# Autodesk Inventor assembly: Trunk
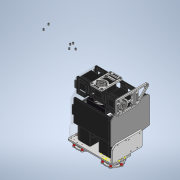
[picture p0: Inventor's stored thumbnail of the model, 180x180]
Saved by Autodesk Inventor 2020.4 (Build 244396000, 396)
## iProperties
Created: 2021-09-10
Part Number: Trunk
Document SubType Name: Assembly
Designer: Masato
Mass: 1170.41 g
Surface Area: 3693.43 cm^2
Volume: 659.985 cm^3
Density: 1.77338 g/cm^3
Author: Masato
## Documents named in this file (20)
- C:\Users\Masato\Documents\Inventor\CIT Brains_Inventor\OpenPlatform_ver3_0 - ve4_1 branch\UpperBody\Trunk\Trunk.iam
- C:\Users\Masato\Documents\Inventor\CIT Brains_Inventor\OpenPlatform_ver3_0 - ve4_1 branch\Ready_Made\KONDO\B3M-SC-1170-A.ipt
- C:\Users\Masato\Documents\Inventor\CIT Brains_Inventor\OpenPlatform_ver3_0 - ve4_1 branch\Ready_Made\KONDO\B3M-SC-1040-A.ipt
- C:\Users\Masato\Documents\Inventor\CIT Brains_Inventor\OpenPlatform_ver3_0 - ve4_1 branch\Ready_Made\Screw\M2_6-15.ipt
- C:\Users\Masato\Documents\Inventor\CIT Brains_Inventor\OpenPlatform_ver3_0 - ve4_1 branch\Ready_Made\KONDO\ClampHorn_Screw.ipt
- C:\Users\Masato\Documents\Inventor\CIT Brains_Inventor\OpenPlatform_ver3_0 - ve4_1 branch\Ready_Made\KONDO\ClampHorn.ipt
- C:\Users\Masato\Documents\Inventor\CIT Brains_Inventor\OpenPlatform_ver3_0 - ve4_1 branch\Ready_Made\Jetson_Xavier_NX_DevKit_without_Wi-FiAntennas\Jetson_Xavier_NX_DevKit.ipt
- C:\Users\Masato\Documents\Inventor\CIT Brains_Inventor\OpenPlatform_ver3_0 - ve4_1 branch\UpperBody\Trunk\Trunk_waisit_frame_.ipt
- C:\Users\Masato\Documents\Inventor\CIT Brains_Inventor\OpenPlatform_ver3_0 - ve4_1 branch\UpperBody\Trunk\CrossRollerBearing\BearingUnit.iam
- C:\Users\Masato\Documents\Inventor\CIT Brains_Inventor\OpenPlatform_ver3_0 - ve4_1 branch\Ready_Made\HP-G830C2800S3.ipt
- C:\Users\Masato\Documents\Inventor\CIT Brains_Inventor\OpenPlatform_ver3_0 - ve4_1 branch\UpperBody\Trunk\Trunk_upper_side_frame.ipt
- C:\Users\Masato\Documents\Inventor\CIT Brains_Inventor\OpenPlatform_ver3_0 - ve4_1 branch\UpperBody\Trunk\Trunk_chest_frame.ipt
- C:\Users\Masato\Documents\Inventor\CIT Brains_Inventor\OpenPlatform_ver3_0 - ve4_1 branch\UpperBody\Trunk\Trunk_lower_side_frame.ipt
- C:\Users\Masato\Documents\Inventor\CIT Brains_Inventor\OpenPlatform_ver3_0 - ve4_1 branch\UpperBody\Trunk\Trunk_shoulder_frame_.ipt
- C:\Users\Masato\Documents\Inventor\CIT Brains_Inventor\OpenPlatform_ver3_0 - ve4_1 branch\UpperBody\Trunk\Trunk_neck_Upper_frame.ipt
- C:\Users\Masato\Documents\Inventor\CIT Brains_Inventor\OpenPlatform_ver3_0 - ve4_1 branch\Ready_Made\InsertNut\IRU-304SW.ipt
- C:\Users\Masato\Documents\Inventor\CIT Brains_Inventor\OpenPlatform_ver3_0 - ve4_1 branch\Ready_Made\Screw\M3-8.ipt
- C:\Users\Masato\Documents\Inventor\CIT Brains_Inventor\OpenPlatform_ver3_0 - ve4_1 branch\UpperBody\Cockpit\Cockpit_side_frame.ipt
- C:\Users\Masato\Documents\Inventor\CIT Brains_Inventor\OpenPlatform_ver3_0 - ve4_1 branch\UpperBody\Cockpit\Cockpit_front_frame.ipt
- ClampHorn.ipt
## Components (48 placed, 19 different names)
1. B3M11xx:3 — 挿入:681, 挿入:686, 挿入:721, 挿入:722
2. B3M-SC-1040-A:4 — 挿入:679, 挿入:684, 挿入:717, 挿入:718, フラッシュ:2, フラッシュ:3
3. B3M-SC-1040-A:5 — 挿入:680, 挿入:685, フラッシュ:2, フラッシュ:3
4. ClampHorn_Screw:3 — 挿入:684
5. ClampHorn_Screw:4 — 挿入:685
6. ClampHorn_Screw:5 — 挿入:686
7. ClampHorn:3 — 挿入:679
8. ClampHorn:4 — 挿入:680
9. ClampHorn:5 — 挿入:681
10. B3M-SC-1170-A:1 — 挿入:689, 挿入:690
11. B3M-SC-1170-A:2 — 挿入:687, 挿入:688
12. Jetson_Xavier_NX_DevKit:1 — フラッシュ:5, フラッシュ:6, メイト:8
13. Trunk_waisit_frame_:1 — フラッシュ:1, 挿入:687, 挿入:688, 挿入:689, 挿入:690, 挿入:693, 挿入:694, 挿入:695, 挿入:696, メイト:5, 挿入:709, 挿入:710, 挿入:711, 挿入:712
14. BearingUnit:1 [sub-assembly] — 挿入:694, 挿入:695
15. BearingUnit:2 [sub-assembly] — 挿入:693, 挿入:696
16. HP-G830C2800S3:1
17. Trunk_upper_side_frame:1 — 挿入:699, 挿入:700, 挿入:713, 挿入:714, 挿入:715, 挿入:716, 挿入:741, 挿入:742, フラッシュ:4, メイト:6
18. Trunk_upper_side_frame:2 — 挿入:701, 挿入:702
19. Trunk_chest_frame:1 — 挿入:699, 挿入:700, 挿入:701, 挿入:702, 挿入:719, 挿入:733, 挿入:734, 挿入:735, 挿入:736, 挿入:737, 挿入:738, 挿入:739, 挿入:740, メイト:7
20. Trunk_lower_side_frame:1 — 挿入:709, 挿入:710, 挿入:713, 挿入:714
21. Trunk_lower_side_frame:2 — 挿入:711, 挿入:712
22. Trunk_shoulder_frame_:1 — 挿入:715, 挿入:716, 挿入:717, 挿入:718
23. Trunk_neck_Upper_frame:1 — 挿入:719, 挿入:721, 挿入:722, 挿入:727, 挿入:728, 挿入:729, 挿入:730, 挿入:731, 挿入:732, 挿入:743, 挿入:744
24. IRU-304SW:1 — 挿入:733
25. IRU-304SW:2 — 挿入:734
26. IRU-304SW:3 — 挿入:735
27. IRU-304SW:4 — 挿入:736
28. IRU-304SW:5 — 挿入:737
29. IRU-304SW:6 — 挿入:738
30. IRU-304SW:7 — 挿入:739
31. IRU-304SW:8 — 挿入:740
32. IRU-304SW:10
33. IRU-304SW:11
34. M3-8:1 — 挿入:728
35. M3-8:2 — 挿入:743
36. M3-8:3 — 挿入:744
37. M3-8:4 — 挿入:727
38. M2_6-15:13 — 挿入:729
39. M2_6-15:14 — 挿入:730
40. M2_6-15:15 — 挿入:731
41. M2_6-15:16 — 挿入:732
42. IRU-304SW:13
43. IRU-304SW:14
44. IRU-304SW:15
45. IRU-304SW:16
46. Trunk_chest_frame:2 — 挿入:741, 挿入:742
47. Cockpit_side_frame:1 — フラッシュ:4, メイト:6, メイト:7, フラッシュ:5, フラッシュ:6, メイト:8, 挿入:745
48. Cockpit_front_frame:1 — 挿入:745
## Relationships (60: Insert 50, Flush 6, Mate 4)
- 挿入:679 [Insert]: B3M-SC-1040-A:4 ↔ ClampHorn:3
- 挿入:680 [Insert]: B3M-SC-1040-A:5 ↔ ClampHorn:4
- 挿入:681 [Insert]: B3M11xx:3 ↔ ClampHorn:5
- 挿入:684 [Insert]: B3M-SC-1040-A:4 ↔ ClampHorn_Screw:3
- 挿入:685 [Insert]: B3M-SC-1040-A:5 ↔ ClampHorn_Screw:4
- 挿入:686 [Insert]: B3M11xx:3 ↔ ClampHorn_Screw:5
- フラッシュ:1 [Flush]: Trunk_waisit_frame_:1
- 挿入:687 [Insert]: B3M-SC-1170-A:2 ↔ Trunk_waisit_frame_:1
- 挿入:688 [Insert]: B3M-SC-1170-A:2 ↔ Trunk_waisit_frame_:1
- 挿入:689 [Insert]: B3M-SC-1170-A:1 ↔ Trunk_waisit_frame_:1
- 挿入:690 [Insert]: B3M-SC-1170-A:1 ↔ Trunk_waisit_frame_:1
- 挿入:693 [Insert]: Trunk_waisit_frame_:1 ↔ BearingUnit:2
- 挿入:694 [Insert]: Trunk_waisit_frame_:1 ↔ BearingUnit:1
- 挿入:695 [Insert]: Trunk_waisit_frame_:1 ↔ BearingUnit:1
- 挿入:696 [Insert]: Trunk_waisit_frame_:1 ↔ BearingUnit:2
- メイト:5 [Mate]: Trunk_waisit_frame_:1
- 挿入:699 [Insert]: Trunk_upper_side_frame:1 ↔ Trunk_chest_frame:1
- 挿入:700 [Insert]: Trunk_upper_side_frame:1 ↔ Trunk_chest_frame:1
- 挿入:701 [Insert]: Trunk_upper_side_frame:2 ↔ Trunk_chest_frame:1
- 挿入:702 [Insert]: Trunk_upper_side_frame:2 ↔ Trunk_chest_frame:1
- 挿入:709 [Insert]: Trunk_waisit_frame_:1 ↔ Trunk_lower_side_frame:1
- 挿入:710 [Insert]: Trunk_waisit_frame_:1 ↔ Trunk_lower_side_frame:1
- 挿入:711 [Insert]: Trunk_waisit_frame_:1 ↔ Trunk_lower_side_frame:2
- 挿入:712 [Insert]: Trunk_waisit_frame_:1 ↔ Trunk_lower_side_frame:2
- 挿入:713 [Insert]: Trunk_upper_side_frame:1 ↔ Trunk_lower_side_frame:1
- 挿入:714 [Insert]: Trunk_upper_side_frame:1 ↔ Trunk_lower_side_frame:1
- 挿入:715 [Insert]: Trunk_upper_side_frame:1 ↔ Trunk_shoulder_frame_:1
- 挿入:716 [Insert]: Trunk_upper_side_frame:1 ↔ Trunk_shoulder_frame_:1
- 挿入:717 [Insert]: B3M-SC-1040-A:4 ↔ Trunk_shoulder_frame_:1
- 挿入:718 [Insert]: B3M-SC-1040-A:4 ↔ Trunk_shoulder_frame_:1
- 挿入:719 [Insert]: Trunk_chest_frame:1 ↔ Trunk_neck_Upper_frame:1
- 挿入:721 [Insert]: B3M11xx:3 ↔ Trunk_neck_Upper_frame:1
- 挿入:722 [Insert]: B3M11xx:3 ↔ Trunk_neck_Upper_frame:1
- 挿入:727 [Insert]: Trunk_neck_Upper_frame:1 ↔ M3-8:4
- 挿入:728 [Insert]: Trunk_neck_Upper_frame:1 ↔ M3-8:1
- 挿入:729 [Insert]: Trunk_neck_Upper_frame:1 ↔ M2_6-15:13
- 挿入:730 [Insert]: Trunk_neck_Upper_frame:1 ↔ M2_6-15:14
- 挿入:731 [Insert]: Trunk_neck_Upper_frame:1 ↔ M2_6-15:15
- 挿入:732 [Insert]: Trunk_neck_Upper_frame:1 ↔ M2_6-15:16
- 挿入:733 [Insert]: Trunk_chest_frame:1 ↔ IRU-304SW:1
- 挿入:734 [Insert]: Trunk_chest_frame:1 ↔ IRU-304SW:2
- 挿入:735 [Insert]: Trunk_chest_frame:1 ↔ IRU-304SW:3
- 挿入:736 [Insert]: Trunk_chest_frame:1 ↔ IRU-304SW:4
- 挿入:737 [Insert]: Trunk_chest_frame:1 ↔ IRU-304SW:5
- 挿入:738 [Insert]: Trunk_chest_frame:1 ↔ IRU-304SW:6
- 挿入:739 [Insert]: Trunk_chest_frame:1 ↔ IRU-304SW:7
- 挿入:740 [Insert]: Trunk_chest_frame:1 ↔ IRU-304SW:8
- 挿入:741 [Insert]: Trunk_upper_side_frame:1 ↔ Trunk_chest_frame:2
- 挿入:742 [Insert]: Trunk_upper_side_frame:1 ↔ Trunk_chest_frame:2
- フラッシュ:2 [Flush]: B3M-SC-1040-A:4 ↔ B3M-SC-1040-A:5
- フラッシュ:3 [Flush]: B3M-SC-1040-A:4 ↔ B3M-SC-1040-A:5
- 挿入:743 [Insert]: Trunk_neck_Upper_frame:1 ↔ M3-8:2
- 挿入:744 [Insert]: Trunk_neck_Upper_frame:1 ↔ M3-8:3
- フラッシュ:4 [Flush]: Trunk_upper_side_frame:1 ↔ Cockpit_side_frame:1
- メイト:6 [Mate]: Trunk_upper_side_frame:1 ↔ Cockpit_side_frame:1
- メイト:7 [Mate] (0.5 mm): Trunk_chest_frame:1 ↔ Cockpit_side_frame:1
- フラッシュ:5 [Flush] (5.05 mm): Jetson_Xavier_NX_DevKit:1 ↔ Cockpit_side_frame:1
- フラッシュ:6 [Flush] (5.05 mm): Jetson_Xavier_NX_DevKit:1 ↔ Cockpit_side_frame:1
- メイト:8 [Mate] (5.5 mm): Jetson_Xavier_NX_DevKit:1 ↔ Cockpit_side_frame:1
- 挿入:745 [Insert]: Cockpit_side_frame:1 ↔ Cockpit_front_frame:1
